(part 1 of 2)
# Autodesk Inventor assembly: Raspberry Pi 3
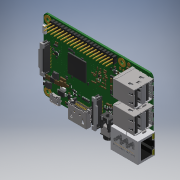
[picture p0: Inventor's stored thumbnail of the model, 180x180]
Saved by Autodesk Inventor 2017 (Build 210142000, 142)
## iProperties
Created: 2016-07-31
Part Number: Raspberry Pi 3
Document SubType Name: Assembly
Designer: jferner
Author: jferner
Sending System: SolidWorks 2016
Last Author: awillame
Last Saved: 2017-12-17
## Documents named in this file (329)
- C:\Users\jferner\Downloads\raspberry-pi-3-model-b-reference-design-solidworks-cad-rpi-raspberrypi-raspberry-pi-1.snapshot.83\Solidworks Complete Assembly\Raspberry Pi 3.iam
- C:\Users\jferner\Downloads\raspberry-pi-3-model-b-reference-design-solidworks-cad-rpi-raspberrypi-raspberry-pi-1.snapshot.83\Solidworks Complete Assembly\Raspberry Pi 3157.ipt
- C:\Users\jferner\Downloads\raspberry-pi-3-model-b-reference-design-solidworks-cad-rpi-raspberrypi-raspberry-pi-1.snapshot.83\Solidworks Complete Assembly\Raspberry Pi 3242.ipt
- C:\Users\jferner\Downloads\raspberry-pi-3-model-b-reference-design-solidworks-cad-rpi-raspberrypi-raspberry-pi-1.snapshot.83\Solidworks Complete Assembly\Raspberry Pi 3266.ipt
- C:\Users\jferner\Downloads\raspberry-pi-3-model-b-reference-design-solidworks-cad-rpi-raspberrypi-raspberry-pi-1.snapshot.83\Solidworks Complete Assembly\raspberry_pi_3(bar_180_2x20).ipt
- C:\Users\jferner\Downloads\raspberry-pi-3-model-b-reference-design-solidworks-cad-rpi-raspberrypi-raspberry-pi-1.snapshot.83\Solidworks Complete Assembly\RPi3_ModelB v1.iam
- C:\Users\jferner\Downloads\raspberry-pi-3-model-b-reference-design-solidworks-cad-rpi-raspberrypi-raspberry-pi-1.snapshot.83\Solidworks Complete Assembly\Raspberry Pi 312.ipt
- C:\Users\jferner\Downloads\raspberry-pi-3-model-b-reference-design-solidworks-cad-rpi-raspberrypi-raspberry-pi-1.snapshot.83\Solidworks Complete Assembly\Raspberry Pi 314.ipt
- C:\Users\jferner\Downloads\raspberry-pi-3-model-b-reference-design-solidworks-cad-rpi-raspberrypi-raspberry-pi-1.snapshot.83\Solidworks Complete Assembly\Raspberry Pi 3172.ipt
- C:\Users\jferner\Downloads\raspberry-pi-3-model-b-reference-design-solidworks-cad-rpi-raspberrypi-raspberry-pi-1.snapshot.83\Solidworks Complete Assembly\Raspberry Pi 3173.ipt
- C:\Users\jferner\Downloads\raspberry-pi-3-model-b-reference-design-solidworks-cad-rpi-raspberrypi-raspberry-pi-1.snapshot.83\Solidworks Complete Assembly\Raspberry Pi 3174.ipt
- C:\Users\jferner\Downloads\raspberry-pi-3-model-b-reference-design-solidworks-cad-rpi-raspberrypi-raspberry-pi-1.snapshot.83\Solidworks Complete Assembly\Raspberry Pi 3175.ipt
- C:\Users\jferner\Downloads\raspberry-pi-3-model-b-reference-design-solidworks-cad-rpi-raspberrypi-raspberry-pi-1.snapshot.83\Solidworks Complete Assembly\Raspberry Pi 3176.ipt
- C:\Users\jferner\Downloads\raspberry-pi-3-model-b-reference-design-solidworks-cad-rpi-raspberrypi-raspberry-pi-1.snapshot.83\Solidworks Complete Assembly\Raspberry Pi 3177.ipt
- C:\Users\jferner\Downloads\raspberry-pi-3-model-b-reference-design-solidworks-cad-rpi-raspberrypi-raspberry-pi-1.snapshot.83\Solidworks Complete Assembly\Raspberry Pi 3178.ipt
- C:\Users\jferner\Downloads\raspberry-pi-3-model-b-reference-design-solidworks-cad-rpi-raspberrypi-raspberry-pi-1.snapshot.83\Solidworks Complete Assembly\Raspberry Pi 3179.ipt
- C:\Users\jferner\Downloads\raspberry-pi-3-model-b-reference-design-solidworks-cad-rpi-raspberrypi-raspberry-pi-1.snapshot.83\Solidworks Complete Assembly\Raspberry Pi 3180.ipt
- C:\Users\jferner\Downloads\raspberry-pi-3-model-b-reference-design-solidworks-cad-rpi-raspberrypi-raspberry-pi-1.snapshot.83\Solidworks Complete Assembly\Raspberry Pi 3181.ipt
- C:\Users\jferner\Downloads\raspberry-pi-3-model-b-reference-design-solidworks-cad-rpi-raspberrypi-raspberry-pi-1.snapshot.83\Solidworks Complete Assembly\Raspberry Pi 3182.ipt
- C:\Users\jferner\Downloads\raspberry-pi-3-model-b-reference-design-solidworks-cad-rpi-raspberrypi-raspberry-pi-1.snapshot.83\Solidworks Complete Assembly\Raspberry Pi 3183.ipt
- C:\Users\jferner\Downloads\raspberry-pi-3-model-b-reference-design-solidworks-cad-rpi-raspberrypi-raspberry-pi-1.snapshot.83\Solidworks Complete Assembly\Raspberry Pi 3184.ipt
- C:\Users\jferner\Downloads\raspberry-pi-3-model-b-reference-design-solidworks-cad-rpi-raspberrypi-raspberry-pi-1.snapshot.83\Solidworks Complete Assembly\Raspberry Pi 3185.ipt
- C:\Users\jferner\Downloads\raspberry-pi-3-model-b-reference-design-solidworks-cad-rpi-raspberrypi-raspberry-pi-1.snapshot.83\Solidworks Complete Assembly\Raspberry Pi 3186.ipt
- C:\Users\jferner\Downloads\raspberry-pi-3-model-b-reference-design-solidworks-cad-rpi-raspberrypi-raspberry-pi-1.snapshot.83\Solidworks Complete Assembly\Raspberry Pi 3187.ipt
- C:\Users\jferner\Downloads\raspberry-pi-3-model-b-reference-design-solidworks-cad-rpi-raspberrypi-raspberry-pi-1.snapshot.83\Solidworks Complete Assembly\Raspberry Pi 3188.ipt
- C:\Users\jferner\Downloads\raspberry-pi-3-model-b-reference-design-solidworks-cad-rpi-raspberrypi-raspberry-pi-1.snapshot.83\Solidworks Complete Assembly\Raspberry Pi 3189.ipt
- C:\Users\jferner\Downloads\raspberry-pi-3-model-b-reference-design-solidworks-cad-rpi-raspberrypi-raspberry-pi-1.snapshot.83\Solidworks Complete Assembly\Raspberry Pi 3190.ipt
- C:\Users\jferner\Downloads\raspberry-pi-3-model-b-reference-design-solidworks-cad-rpi-raspberrypi-raspberry-pi-1.snapshot.83\Solidworks Complete Assembly\Raspberry Pi 3191.ipt
- C:\Users\jferner\Downloads\raspberry-pi-3-model-b-reference-design-solidworks-cad-rpi-raspberrypi-raspberry-pi-1.snapshot.83\Solidworks Complete Assembly\Raspberry Pi 3192.ipt
- C:\Users\jferner\Downloads\raspberry-pi-3-model-b-reference-design-solidworks-cad-rpi-raspberrypi-raspberry-pi-1.snapshot.83\Solidworks Complete Assembly\Raspberry Pi 3193.ipt
- C:\Users\jferner\Downloads\raspberry-pi-3-model-b-reference-design-solidworks-cad-rpi-raspberrypi-raspberry-pi-1.snapshot.83\Solidworks Complete Assembly\Raspberry Pi 3194.ipt
- C:\Users\jferner\Downloads\raspberry-pi-3-model-b-reference-design-solidworks-cad-rpi-raspberrypi-raspberry-pi-1.snapshot.83\Solidworks Complete Assembly\Raspberry Pi 3195.ipt
- C:\Users\jferner\Downloads\raspberry-pi-3-model-b-reference-design-solidworks-cad-rpi-raspberrypi-raspberry-pi-1.snapshot.83\Solidworks Complete Assembly\Raspberry Pi 3196.ipt
- C:\Users\jferner\Downloads\raspberry-pi-3-model-b-reference-design-solidworks-cad-rpi-raspberrypi-raspberry-pi-1.snapshot.83\Solidworks Complete Assembly\Raspberry Pi 3197.ipt
- C:\Users\jferner\Downloads\raspberry-pi-3-model-b-reference-design-solidworks-cad-rpi-raspberrypi-raspberry-pi-1.snapshot.83\Solidworks Complete Assembly\Raspberry Pi 3198.ipt
- C:\Users\jferner\Downloads\raspberry-pi-3-model-b-reference-design-solidworks-cad-rpi-raspberrypi-raspberry-pi-1.snapshot.83\Solidworks Complete Assembly\Raspberry Pi 3199.ipt
- C:\Users\jferner\Downloads\raspberry-pi-3-model-b-reference-design-solidworks-cad-rpi-raspberrypi-raspberry-pi-1.snapshot.83\Solidworks Complete Assembly\Raspberry Pi 3200.ipt
- C:\Users\jferner\Downloads\raspberry-pi-3-model-b-reference-design-solidworks-cad-rpi-raspberrypi-raspberry-pi-1.snapshot.83\Solidworks Complete Assembly\Raspberry Pi 3201.ipt
- C:\Users\jferner\Downloads\raspberry-pi-3-model-b-reference-design-solidworks-cad-rpi-raspberrypi-raspberry-pi-1.snapshot.83\Solidworks Complete Assembly\Raspberry Pi 3202.ipt
- C:\Users\jferner\Downloads\raspberry-pi-3-model-b-reference-design-solidworks-cad-rpi-raspberrypi-raspberry-pi-1.snapshot.83\Solidworks Complete Assembly\Raspberry Pi 3203.ipt
- C:\Users\jferner\Downloads\raspberry-pi-3-model-b-reference-design-solidworks-cad-rpi-raspberrypi-raspberry-pi-1.snapshot.83\Solidworks Complete Assembly\Raspberry Pi 3204.ipt
- C:\Users\jferner\Downloads\raspberry-pi-3-model-b-reference-design-solidworks-cad-rpi-raspberrypi-raspberry-pi-1.snapshot.83\Solidworks Complete Assembly\Raspberry Pi 3205.ipt
- C:\Users\jferner\Downloads\raspberry-pi-3-model-b-reference-design-solidworks-cad-rpi-raspberrypi-raspberry-pi-1.snapshot.83\Solidworks Complete Assembly\Raspberry Pi 3206.ipt
- C:\Users\jferner\Downloads\raspberry-pi-3-model-b-reference-design-solidworks-cad-rpi-raspberrypi-raspberry-pi-1.snapshot.83\Solidworks Complete Assembly\Raspberry Pi 3207.ipt
- C:\Users\jferner\Downloads\raspberry-pi-3-model-b-reference-design-solidworks-cad-rpi-raspberrypi-raspberry-pi-1.snapshot.83\Solidworks Complete Assembly\Raspberry Pi 3208.ipt
- C:\Users\jferner\Downloads\raspberry-pi-3-model-b-reference-design-solidworks-cad-rpi-raspberrypi-raspberry-pi-1.snapshot.83\Solidworks Complete Assembly\Raspberry Pi 3209.ipt
- C:\Users\jferner\Downloads\raspberry-pi-3-model-b-reference-design-solidworks-cad-rpi-raspberrypi-raspberry-pi-1.snapshot.83\Solidworks Complete Assembly\Raspberry Pi 3210.ipt
- C:\Users\jferner\Downloads\raspberry-pi-3-model-b-reference-design-solidworks-cad-rpi-raspberrypi-raspberry-pi-1.snapshot.83\Solidworks Complete Assembly\Raspberry Pi 3211.ipt
- C:\Users\jferner\Downloads\raspberry-pi-3-model-b-reference-design-solidworks-cad-rpi-raspberrypi-raspberry-pi-1.snapshot.83\Solidworks Complete Assembly\Raspberry Pi 3212.ipt
- C:\Users\jferner\Downloads\raspberry-pi-3-model-b-reference-design-solidworks-cad-rpi-raspberrypi-raspberry-pi-1.snapshot.83\Solidworks Complete Assembly\Raspberry Pi 3213.ipt
- C:\Users\jferner\Downloads\raspberry-pi-3-model-b-reference-design-solidworks-cad-rpi-raspberrypi-raspberry-pi-1.snapshot.83\Solidworks Complete Assembly\Raspberry Pi 3214.ipt
- C:\Users\jferner\Downloads\raspberry-pi-3-model-b-reference-design-solidworks-cad-rpi-raspberrypi-raspberry-pi-1.snapshot.83\Solidworks Complete Assembly\Raspberry Pi 3215.ipt
- C:\Users\jferner\Downloads\raspberry-pi-3-model-b-reference-design-solidworks-cad-rpi-raspberrypi-raspberry-pi-1.snapshot.83\Solidworks Complete Assembly\Raspberry Pi 3216.ipt
- C:\Users\jferner\Downloads\raspberry-pi-3-model-b-reference-design-solidworks-cad-rpi-raspberrypi-raspberry-pi-1.snapshot.83\Solidworks Complete Assembly\Raspberry Pi 3217.ipt
- C:\Users\jferner\Downloads\raspberry-pi-3-model-b-reference-design-solidworks-cad-rpi-raspberrypi-raspberry-pi-1.snapshot.83\Solidworks Complete Assembly\Raspberry Pi 3218.ipt
- C:\Users\jferner\Downloads\raspberry-pi-3-model-b-reference-design-solidworks-cad-rpi-raspberrypi-raspberry-pi-1.snapshot.83\Solidworks Complete Assembly\Raspberry Pi 3219.ipt
- C:\Users\jferner\Downloads\raspberry-pi-3-model-b-reference-design-solidworks-cad-rpi-raspberrypi-raspberry-pi-1.snapshot.83\Solidworks Complete Assembly\Raspberry Pi 3220.ipt
- C:\Users\jferner\Downloads\raspberry-pi-3-model-b-reference-design-solidworks-cad-rpi-raspberrypi-raspberry-pi-1.snapshot.83\Solidworks Complete Assembly\Raspberry Pi 3221.ipt
- C:\Users\jferner\Downloads\raspberry-pi-3-model-b-reference-design-solidworks-cad-rpi-raspberrypi-raspberry-pi-1.snapshot.83\Solidworks Complete Assembly\Raspberry Pi 3222.ipt
- C:\Users\jferner\Downloads\raspberry-pi-3-model-b-reference-design-solidworks-cad-rpi-raspberrypi-raspberry-pi-1.snapshot.83\Solidworks Complete Assembly\Raspberry Pi 3223.ipt
- C:\Users\jferner\Downloads\raspberry-pi-3-model-b-reference-design-solidworks-cad-rpi-raspberrypi-raspberry-pi-1.snapshot.83\Solidworks Complete Assembly\Raspberry Pi 3224.ipt
- C:\Users\jferner\Downloads\raspberry-pi-3-model-b-reference-design-solidworks-cad-rpi-raspberrypi-raspberry-pi-1.snapshot.83\Solidworks Complete Assembly\Raspberry Pi 3225.ipt
- C:\Users\jferner\Downloads\raspberry-pi-3-model-b-reference-design-solidworks-cad-rpi-raspberrypi-raspberry-pi-1.snapshot.83\Solidworks Complete Assembly\Raspberry Pi 3226.ipt
- C:\Users\jferner\Downloads\raspberry-pi-3-model-b-reference-design-solidworks-cad-rpi-raspberrypi-raspberry-pi-1.snapshot.83\Solidworks Complete Assembly\Raspberry Pi 3227.ipt
- C:\Users\jferner\Downloads\raspberry-pi-3-model-b-reference-design-solidworks-cad-rpi-raspberrypi-raspberry-pi-1.snapshot.83\Solidworks Complete Assembly\Raspberry Pi 3228.ipt
- C:\Users\jferner\Downloads\raspberry-pi-3-model-b-reference-design-solidworks-cad-rpi-raspberrypi-raspberry-pi-1.snapshot.83\Solidworks Complete Assembly\Raspberry Pi 3229.ipt
- C:\Users\jferner\Downloads\raspberry-pi-3-model-b-reference-design-solidworks-cad-rpi-raspberrypi-raspberry-pi-1.snapshot.83\Solidworks Complete Assembly\Raspberry Pi 3230.ipt
- C:\Users\jferner\Downloads\raspberry-pi-3-model-b-reference-design-solidworks-cad-rpi-raspberrypi-raspberry-pi-1.snapshot.83\Solidworks Complete Assembly\Raspberry Pi 3231.ipt
- C:\Users\jferner\Downloads\raspberry-pi-3-model-b-reference-design-solidworks-cad-rpi-raspberrypi-raspberry-pi-1.snapshot.83\Solidworks Complete Assembly\Raspberry Pi 3232.ipt
- C:\Users\jferner\Downloads\raspberry-pi-3-model-b-reference-design-solidworks-cad-rpi-raspberrypi-raspberry-pi-1.snapshot.83\Solidworks Complete Assembly\Raspberry Pi 3233.ipt
- C:\Users\jferner\Downloads\raspberry-pi-3-model-b-reference-design-solidworks-cad-rpi-raspberrypi-raspberry-pi-1.snapshot.83\Solidworks Complete Assembly\Raspberry Pi 3234.ipt
- C:\Users\jferner\Downloads\raspberry-pi-3-model-b-reference-design-solidworks-cad-rpi-raspberrypi-raspberry-pi-1.snapshot.83\Solidworks Complete Assembly\Raspberry Pi 3235.ipt
- C:\Users\jferner\Downloads\raspberry-pi-3-model-b-reference-design-solidworks-cad-rpi-raspberrypi-raspberry-pi-1.snapshot.83\Solidworks Complete Assembly\Raspberry Pi 31.ipt
- C:\Users\jferner\Downloads\raspberry-pi-3-model-b-reference-design-solidworks-cad-rpi-raspberrypi-raspberry-pi-1.snapshot.83\Solidworks Complete Assembly\Raspberry Pi 36.ipt
- C:\Users\jferner\Downloads\raspberry-pi-3-model-b-reference-design-solidworks-cad-rpi-raspberrypi-raspberry-pi-1.snapshot.83\Solidworks Complete Assembly\Raspberry Pi 32.ipt
- C:\Users\jferner\Downloads\raspberry-pi-3-model-b-reference-design-solidworks-cad-rpi-raspberrypi-raspberry-pi-1.snapshot.83\Solidworks Complete Assembly\Raspberry Pi 33.ipt
- C:\Users\jferner\Downloads\raspberry-pi-3-model-b-reference-design-solidworks-cad-rpi-raspberrypi-raspberry-pi-1.snapshot.83\Solidworks Complete Assembly\Raspberry Pi 34.ipt
- C:\Users\jferner\Downloads\raspberry-pi-3-model-b-reference-design-solidworks-cad-rpi-raspberrypi-raspberry-pi-1.snapshot.83\Solidworks Complete Assembly\Raspberry Pi 35.ipt
- C:\Users\jferner\Downloads\raspberry-pi-3-model-b-reference-design-solidworks-cad-rpi-raspberrypi-raspberry-pi-1.snapshot.83\Solidworks Complete Assembly\Raspberry Pi 37.ipt
- C:\Users\jferner\Downloads\raspberry-pi-3-model-b-reference-design-solidworks-cad-rpi-raspberrypi-raspberry-pi-1.snapshot.83\Solidworks Complete Assembly\Raspberry Pi 38.ipt
- C:\Users\jferner\Downloads\raspberry-pi-3-model-b-reference-design-solidworks-cad-rpi-raspberrypi-raspberry-pi-1.snapshot.83\Solidworks Complete Assembly\Raspberry Pi 39.ipt
- C:\Users\jferner\Downloads\raspberry-pi-3-model-b-reference-design-solidworks-cad-rpi-raspberrypi-raspberry-pi-1.snapshot.83\Solidworks Complete Assembly\Raspberry Pi 310.ipt
- C:\Users\jferner\Downloads\raspberry-pi-3-model-b-reference-design-solidworks-cad-rpi-raspberrypi-raspberry-pi-1.snapshot.83\Solidworks Complete Assembly\Raspberry Pi 311.ipt
- C:\Users\jferner\Downloads\raspberry-pi-3-model-b-reference-design-solidworks-cad-rpi-raspberrypi-raspberry-pi-1.snapshot.83\Solidworks Complete Assembly\Raspberry Pi 313.ipt
- C:\Users\jferner\Downloads\raspberry-pi-3-model-b-reference-design-solidworks-cad-rpi-raspberrypi-raspberry-pi-1.snapshot.83\Solidworks Complete Assembly\Raspberry Pi 315.ipt
- C:\Users\jferner\Downloads\raspberry-pi-3-model-b-reference-design-solidworks-cad-rpi-raspberrypi-raspberry-pi-1.snapshot.83\Solidworks Complete Assembly\Raspberry Pi 316.ipt
- C:\Users\jferner\Downloads\raspberry-pi-3-model-b-reference-design-solidworks-cad-rpi-raspberrypi-raspberry-pi-1.snapshot.83\Solidworks Complete Assembly\Raspberry Pi 317.ipt
- C:\Users\jferner\Downloads\raspberry-pi-3-model-b-reference-design-solidworks-cad-rpi-raspberrypi-raspberry-pi-1.snapshot.83\Solidworks Complete Assembly\Raspberry Pi 318.ipt
- C:\Users\jferner\Downloads\raspberry-pi-3-model-b-reference-design-solidworks-cad-rpi-raspberrypi-raspberry-pi-1.snapshot.83\Solidworks Complete Assembly\Raspberry Pi 319.ipt
- C:\Users\jferner\Downloads\raspberry-pi-3-model-b-reference-design-solidworks-cad-rpi-raspberrypi-raspberry-pi-1.snapshot.83\Solidworks Complete Assembly\Raspberry Pi 320.ipt
- C:\Users\jferner\Downloads\raspberry-pi-3-model-b-reference-design-solidworks-cad-rpi-raspberrypi-raspberry-pi-1.snapshot.83\Solidworks Complete Assembly\Raspberry Pi 322.ipt
- C:\Users\jferner\Downloads\raspberry-pi-3-model-b-reference-design-solidworks-cad-rpi-raspberrypi-raspberry-pi-1.snapshot.83\Solidworks Complete Assembly\Raspberry Pi 323.ipt
- C:\Users\jferner\Downloads\raspberry-pi-3-model-b-reference-design-solidworks-cad-rpi-raspberrypi-raspberry-pi-1.snapshot.83\Solidworks Complete Assembly\Raspberry Pi 324.ipt
- C:\Users\jferner\Downloads\raspberry-pi-3-model-b-reference-design-solidworks-cad-rpi-raspberrypi-raspberry-pi-1.snapshot.83\Solidworks Complete Assembly\Raspberry Pi 325.ipt
- C:\Users\jferner\Downloads\raspberry-pi-3-model-b-reference-design-solidworks-cad-rpi-raspberrypi-raspberry-pi-1.snapshot.83\Solidworks Complete Assembly\Raspberry Pi 326.ipt
- C:\Users\jferner\Downloads\raspberry-pi-3-model-b-reference-design-solidworks-cad-rpi-raspberrypi-raspberry-pi-1.snapshot.83\Solidworks Complete Assembly\Raspberry Pi 327.ipt
- C:\Users\jferner\Downloads\raspberry-pi-3-model-b-reference-design-solidworks-cad-rpi-raspberrypi-raspberry-pi-1.snapshot.83\Solidworks Complete Assembly\Raspberry Pi 328.ipt
- C:\Users\jferner\Downloads\raspberry-pi-3-model-b-reference-design-solidworks-cad-rpi-raspberrypi-raspberry-pi-1.snapshot.83\Solidworks Complete Assembly\Raspberry Pi 329.ipt
- C:\Users\jferner\Downloads\raspberry-pi-3-model-b-reference-design-solidworks-cad-rpi-raspberrypi-raspberry-pi-1.snapshot.83\Solidworks Complete Assembly\Raspberry Pi 330.ipt
- C:\Users\jferner\Downloads\raspberry-pi-3-model-b-reference-design-solidworks-cad-rpi-raspberrypi-raspberry-pi-1.snapshot.83\Solidworks Complete Assembly\Raspberry Pi 331.ipt
- C:\Users\jferner\Downloads\raspberry-pi-3-model-b-reference-design-solidworks-cad-rpi-raspberrypi-raspberry-pi-1.snapshot.83\Solidworks Complete Assembly\Raspberry Pi 332.ipt
- C:\Users\jferner\Downloads\raspberry-pi-3-model-b-reference-design-solidworks-cad-rpi-raspberrypi-raspberry-pi-1.snapshot.83\Solidworks Complete Assembly\Raspberry Pi 333.ipt
- C:\Users\jferner\Downloads\raspberry-pi-3-model-b-reference-design-solidworks-cad-rpi-raspberrypi-raspberry-pi-1.snapshot.83\Solidworks Complete Assembly\Raspberry Pi 334.ipt
- C:\Users\jferner\Downloads\raspberry-pi-3-model-b-reference-design-solidworks-cad-rpi-raspberrypi-raspberry-pi-1.snapshot.83\Solidworks Complete Assembly\Raspberry Pi 335.ipt
- C:\Users\jferner\Downloads\raspberry-pi-3-model-b-reference-design-solidworks-cad-rpi-raspberrypi-raspberry-pi-1.snapshot.83\Solidworks Complete Assembly\Raspberry Pi 336.ipt
- C:\Users\jferner\Downloads\raspberry-pi-3-model-b-reference-design-solidworks-cad-rpi-raspberrypi-raspberry-pi-1.snapshot.83\Solidworks Complete Assembly\Raspberry Pi 337.ipt
- C:\Users\jferner\Downloads\raspberry-pi-3-model-b-reference-design-solidworks-cad-rpi-raspberrypi-raspberry-pi-1.snapshot.83\Solidworks Complete Assembly\Raspberry Pi 338.ipt
- C:\Users\jferner\Downloads\raspberry-pi-3-model-b-reference-design-solidworks-cad-rpi-raspberrypi-raspberry-pi-1.snapshot.83\Solidworks Complete Assembly\Raspberry Pi 339.ipt
- C:\Users\jferner\Downloads\raspberry-pi-3-model-b-reference-design-solidworks-cad-rpi-raspberrypi-raspberry-pi-1.snapshot.83\Solidworks Complete Assembly\Raspberry Pi 340.ipt
- C:\Users\jferner\Downloads\raspberry-pi-3-model-b-reference-design-solidworks-cad-rpi-raspberrypi-raspberry-pi-1.snapshot.83\Solidworks Complete Assembly\Raspberry Pi 341.ipt
- C:\Users\jferner\Downloads\raspberry-pi-3-model-b-reference-design-solidworks-cad-rpi-raspberrypi-raspberry-pi-1.snapshot.83\Solidworks Complete Assembly\Raspberry Pi 342.ipt
- C:\Users\jferner\Downloads\raspberry-pi-3-model-b-reference-design-solidworks-cad-rpi-raspberrypi-raspberry-pi-1.snapshot.83\Solidworks Complete Assembly\Raspberry Pi 343.ipt
- C:\Users\jferner\Downloads\raspberry-pi-3-model-b-reference-design-solidworks-cad-rpi-raspberrypi-raspberry-pi-1.snapshot.83\Solidworks Complete Assembly\Raspberry Pi 344.ipt
- C:\Users\jferner\Downloads\raspberry-pi-3-model-b-reference-design-solidworks-cad-rpi-raspberrypi-raspberry-pi-1.snapshot.83\Solidworks Complete Assembly\Raspberry Pi 345.ipt
- C:\Users\jferner\Downloads\raspberry-pi-3-model-b-reference-design-solidworks-cad-rpi-raspberrypi-raspberry-pi-1.snapshot.83\Solidworks Complete Assembly\Raspberry Pi 346.ipt
- C:\Users\jferner\Downloads\raspberry-pi-3-model-b-reference-design-solidworks-cad-rpi-raspberrypi-raspberry-pi-1.snapshot.83\Solidworks Complete Assembly\Raspberry Pi 347.ipt
- C:\Users\jferner\Downloads\raspberry-pi-3-model-b-reference-design-solidworks-cad-rpi-raspberrypi-raspberry-pi-1.snapshot.83\Solidworks Complete Assembly\Raspberry Pi 348.ipt
- C:\Users\jferner\Downloads\raspberry-pi-3-model-b-reference-design-solidworks-cad-rpi-raspberrypi-raspberry-pi-1.snapshot.83\Solidworks Complete Assembly\Raspberry Pi 349.ipt
- C:\Users\jferner\Downloads\raspberry-pi-3-model-b-reference-design-solidworks-cad-rpi-raspberrypi-raspberry-pi-1.snapshot.83\Solidworks Complete Assembly\Raspberry Pi 350.ipt
- C:\Users\jferner\Downloads\raspberry-pi-3-model-b-reference-design-solidworks-cad-rpi-raspberrypi-raspberry-pi-1.snapshot.83\Solidworks Complete Assembly\Raspberry Pi 351.ipt
- C:\Users\jferner\Downloads\raspberry-pi-3-model-b-reference-design-solidworks-cad-rpi-raspberrypi-raspberry-pi-1.snapshot.83\Solidworks Complete Assembly\Raspberry Pi 352.ipt
- C:\Users\jferner\Downloads\raspberry-pi-3-model-b-reference-design-solidworks-cad-rpi-raspberrypi-raspberry-pi-1.snapshot.83\Solidworks Complete Assembly\Raspberry Pi 353.ipt
- C:\Users\jferner\Downloads\raspberry-pi-3-model-b-reference-design-solidworks-cad-rpi-raspberrypi-raspberry-pi-1.snapshot.83\Solidworks Complete Assembly\Raspberry Pi 354.ipt
- C:\Users\jferner\Downloads\raspberry-pi-3-model-b-reference-design-solidworks-cad-rpi-raspberrypi-raspberry-pi-1.snapshot.83\Solidworks Complete Assembly\Raspberry Pi 355.ipt
- C:\Users\jferner\Downloads\raspberry-pi-3-model-b-reference-design-solidworks-cad-rpi-raspberrypi-raspberry-pi-1.snapshot.83\Solidworks Complete Assembly\Raspberry Pi 356.ipt
- C:\Users\jferner\Downloads\raspberry-pi-3-model-b-reference-design-solidworks-cad-rpi-raspberrypi-raspberry-pi-1.snapshot.83\Solidworks Complete Assembly\Raspberry Pi 357.ipt
- C:\Users\jferner\Downloads\raspberry-pi-3-model-b-reference-design-solidworks-cad-rpi-raspberrypi-raspberry-pi-1.snapshot.83\Solidworks Complete Assembly\Raspberry Pi 358.ipt
- C:\Users\jferner\Downloads\raspberry-pi-3-model-b-reference-design-solidworks-cad-rpi-raspberrypi-raspberry-pi-1.snapshot.83\Solidworks Complete Assembly\Raspberry Pi 359.ipt
- C:\Users\jferner\Downloads\raspberry-pi-3-model-b-reference-design-solidworks-cad-rpi-raspberrypi-raspberry-pi-1.snapshot.83\Solidworks Complete Assembly\Raspberry Pi 360.ipt
- C:\Users\jferner\Downloads\raspberry-pi-3-model-b-reference-design-solidworks-cad-rpi-raspberrypi-raspberry-pi-1.snapshot.83\Solidworks Complete Assembly\Raspberry Pi 361.ipt
- C:\Users\jferner\Downloads\raspberry-pi-3-model-b-reference-design-solidworks-cad-rpi-raspberrypi-raspberry-pi-1.snapshot.83\Solidworks Complete Assembly\Raspberry Pi 362.ipt
- C:\Users\jferner\Downloads\raspberry-pi-3-model-b-reference-design-solidworks-cad-rpi-raspberrypi-raspberry-pi-1.snapshot.83\Solidworks Complete Assembly\Raspberry Pi 363.ipt
- C:\Users\jferner\Downloads\raspberry-pi-3-model-b-reference-design-solidworks-cad-rpi-raspberrypi-raspberry-pi-1.snapshot.83\Solidworks Complete Assembly\Raspberry Pi 364.ipt
- C:\Users\jferner\Downloads\raspberry-pi-3-model-b-reference-design-solidworks-cad-rpi-raspberrypi-raspberry-pi-1.snapshot.83\Solidworks Complete Assembly\Raspberry Pi 365.ipt
- C:\Users\jferner\Downloads\raspberry-pi-3-model-b-reference-design-solidworks-cad-rpi-raspberrypi-raspberry-pi-1.snapshot.83\Solidworks Complete Assembly\Raspberry Pi 366.ipt
- C:\Users\jferner\Downloads\raspberry-pi-3-model-b-reference-design-solidworks-cad-rpi-raspberrypi-raspberry-pi-1.snapshot.83\Solidworks Complete Assembly\Raspberry Pi 367.ipt
- C:\Users\jferner\Downloads\raspberry-pi-3-model-b-reference-design-solidworks-cad-rpi-raspberrypi-raspberry-pi-1.snapshot.83\Solidworks Complete Assembly\Raspberry Pi 368.ipt
- C:\Users\jferner\Downloads\raspberry-pi-3-model-b-reference-design-solidworks-cad-rpi-raspberrypi-raspberry-pi-1.snapshot.83\Solidworks Complete Assembly\Raspberry Pi 369.ipt
- C:\Users\jferner\Downloads\raspberry-pi-3-model-b-reference-design-solidworks-cad-rpi-raspberrypi-raspberry-pi-1.snapshot.83\Solidworks Complete Assembly\Raspberry Pi 370.ipt
- C:\Users\jferner\Downloads\raspberry-pi-3-model-b-reference-design-solidworks-cad-rpi-raspberrypi-raspberry-pi-1.snapshot.83\Solidworks Complete Assembly\Raspberry Pi 371.ipt
- C:\Users\jferner\Downloads\raspberry-pi-3-model-b-reference-design-solidworks-cad-rpi-raspberrypi-raspberry-pi-1.snapshot.83\Solidworks Complete Assembly\Raspberry Pi 372.ipt
- C:\Users\jferner\Downloads\raspberry-pi-3-model-b-reference-design-solidworks-cad-rpi-raspberrypi-raspberry-pi-1.snapshot.83\Solidworks Complete Assembly\Raspberry Pi 373.ipt
- C:\Users\jferner\Downloads\raspberry-pi-3-model-b-reference-design-solidworks-cad-rpi-raspberrypi-raspberry-pi-1.snapshot.83\Solidworks Complete Assembly\Raspberry Pi 374.ipt
- C:\Users\jferner\Downloads\raspberry-pi-3-model-b-reference-design-solidworks-cad-rpi-raspberrypi-raspberry-pi-1.snapshot.83\Solidworks Complete Assembly\Raspberry Pi 375.ipt
- C:\Users\jferner\Downloads\raspberry-pi-3-model-b-reference-design-solidworks-cad-rpi-raspberrypi-raspberry-pi-1.snapshot.83\Solidworks Complete Assembly\Raspberry Pi 376.ipt
- C:\Users\jferner\Downloads\raspberry-pi-3-model-b-reference-design-solidworks-cad-rpi-raspberrypi-raspberry-pi-1.snapshot.83\Solidworks Complete Assembly\Raspberry Pi 377.ipt
- C:\Users\jferner\Downloads\raspberry-pi-3-model-b-reference-design-solidworks-cad-rpi-raspberrypi-raspberry-pi-1.snapshot.83\Solidworks Complete Assembly\Raspberry Pi 378.ipt
- C:\Users\jferner\Downloads\raspberry-pi-3-model-b-reference-design-solidworks-cad-rpi-raspberrypi-raspberry-pi-1.snapshot.83\Solidworks Complete Assembly\Raspberry Pi 379.ipt
- C:\Users\jferner\Downloads\raspberry-pi-3-model-b-reference-design-solidworks-cad-rpi-raspberrypi-raspberry-pi-1.snapshot.83\Solidworks Complete Assembly\Raspberry Pi 380.ipt
- C:\Users\jferner\Downloads\raspberry-pi-3-model-b-reference-design-solidworks-cad-rpi-raspberrypi-raspberry-pi-1.snapshot.83\Solidworks Complete Assembly\Raspberry Pi 381.ipt
- C:\Users\jferner\Downloads\raspberry-pi-3-model-b-reference-design-solidworks-cad-rpi-raspberrypi-raspberry-pi-1.snapshot.83\Solidworks Complete Assembly\Raspberry Pi 382.ipt
- C:\Users\jferner\Downloads\raspberry-pi-3-model-b-reference-design-solidworks-cad-rpi-raspberrypi-raspberry-pi-1.snapshot.83\Solidworks Complete Assembly\Raspberry Pi 383.ipt
- C:\Users\jferner\Downloads\raspberry-pi-3-model-b-reference-design-solidworks-cad-rpi-raspberrypi-raspberry-pi-1.snapshot.83\Solidworks Complete Assembly\Raspberry Pi 385.ipt
- C:\Users\jferner\Downloads\raspberry-pi-3-model-b-reference-design-solidworks-cad-rpi-raspberrypi-raspberry-pi-1.snapshot.83\Solidworks Complete Assembly\Raspberry Pi 386.ipt
- C:\Users\jferner\Downloads\raspberry-pi-3-model-b-reference-design-solidworks-cad-rpi-raspberrypi-raspberry-pi-1.snapshot.83\Solidworks Complete Assembly\Raspberry Pi 387.ipt
- C:\Users\jferner\Downloads\raspberry-pi-3-model-b-reference-design-solidworks-cad-rpi-raspberrypi-raspberry-pi-1.snapshot.83\Solidworks Complete Assembly\Raspberry Pi 388.ipt
- C:\Users\jferner\Downloads\raspberry-pi-3-model-b-reference-design-solidworks-cad-rpi-raspberrypi-raspberry-pi-1.snapshot.83\Solidworks Complete Assembly\Raspberry Pi 390.ipt
- C:\Users\jferner\Downloads\raspberry-pi-3-model-b-reference-design-solidworks-cad-rpi-raspberrypi-raspberry-pi-1.snapshot.83\Solidworks Complete Assembly\Raspberry Pi 391.ipt
- C:\Users\jferner\Downloads\raspberry-pi-3-model-b-reference-design-solidworks-cad-rpi-raspberrypi-raspberry-pi-1.snapshot.83\Solidworks Complete Assembly\Raspberry Pi 393.ipt
- C:\Users\jferner\Downloads\raspberry-pi-3-model-b-reference-design-solidworks-cad-rpi-raspberrypi-raspberry-pi-1.snapshot.83\Solidworks Complete Assembly\Raspberry Pi 394.ipt
- C:\Users\jferner\Downloads\raspberry-pi-3-model-b-reference-design-solidworks-cad-rpi-raspberrypi-raspberry-pi-1.snapshot.83\Solidworks Complete Assembly\Raspberry Pi 395.ipt
- C:\Users\jferner\Downloads\raspberry-pi-3-model-b-reference-design-solidworks-cad-rpi-raspberrypi-raspberry-pi-1.snapshot.83\Solidworks Complete Assembly\Raspberry Pi 396.ipt
- C:\Users\jferner\Downloads\raspberry-pi-3-model-b-reference-design-solidworks-cad-rpi-raspberrypi-raspberry-pi-1.snapshot.83\Solidworks Complete Assembly\Raspberry Pi 397.ipt
- C:\Users\jferner\Downloads\raspberry-pi-3-model-b-reference-design-solidworks-cad-rpi-raspberrypi-raspberry-pi-1.snapshot.83\Solidworks Complete Assembly\Raspberry Pi 398.ipt
- C:\Users\jferner\Downloads\raspberry-pi-3-model-b-reference-design-solidworks-cad-rpi-raspberrypi-raspberry-pi-1.snapshot.83\Solidworks Complete Assembly\Raspberry Pi 399.ipt
- C:\Users\jferner\Downloads\raspberry-pi-3-model-b-reference-design-solidworks-cad-rpi-raspberrypi-raspberry-pi-1.snapshot.83\Solidworks Complete Assembly\Raspberry Pi 3100.ipt
- C:\Users\jferner\Downloads\raspberry-pi-3-model-b-reference-design-solidworks-cad-rpi-raspberrypi-raspberry-pi-1.snapshot.83\Solidworks Complete Assembly\Raspberry Pi 3101.ipt
- C:\Users\jferner\Downloads\raspberry-pi-3-model-b-reference-design-solidworks-cad-rpi-raspberrypi-raspberry-pi-1.snapshot.83\Solidworks Complete Assembly\Raspberry Pi 3102.ipt
- C:\Users\jferner\Downloads\raspberry-pi-3-model-b-reference-design-solidworks-cad-rpi-raspberrypi-raspberry-pi-1.snapshot.83\Solidworks Complete Assembly\Raspberry Pi 3103.ipt
- C:\Users\jferner\Downloads\raspberry-pi-3-model-b-reference-design-solidworks-cad-rpi-raspberrypi-raspberry-pi-1.snapshot.83\Solidworks Complete Assembly\Raspberry Pi 3104.ipt
- C:\Users\jferner\Downloads\raspberry-pi-3-model-b-reference-design-solidworks-cad-rpi-raspberrypi-raspberry-pi-1.snapshot.83\Solidworks Complete Assembly\Raspberry Pi 3105.ipt
- C:\Users\jferner\Downloads\raspberry-pi-3-model-b-reference-design-solidworks-cad-rpi-raspberrypi-raspberry-pi-1.snapshot.83\Solidworks Complete Assembly\Raspberry Pi 3106.ipt
- C:\Users\jferner\Downloads\raspberry-pi-3-model-b-reference-design-solidworks-cad-rpi-raspberrypi-raspberry-pi-1.snapshot.83\Solidworks Complete Assembly\Raspberry Pi 3107.ipt
- C:\Users\jferner\Downloads\raspberry-pi-3-model-b-reference-design-solidworks-cad-rpi-raspberrypi-raspberry-pi-1.snapshot.83\Solidworks Complete Assembly\Raspberry Pi 3108.ipt
- C:\Users\jferner\Downloads\raspberry-pi-3-model-b-reference-design-solidworks-cad-rpi-raspberrypi-raspberry-pi-1.snapshot.83\Solidworks Complete Assembly\Raspberry Pi 3109.ipt
- C:\Users\jferner\Downloads\raspberry-pi-3-model-b-reference-design-solidworks-cad-rpi-raspberrypi-raspberry-pi-1.snapshot.83\Solidworks Complete Assembly\Raspberry Pi 3110.ipt
- C:\Users\jferner\Downloads\raspberry-pi-3-model-b-reference-design-solidworks-cad-rpi-raspberrypi-raspberry-pi-1.snapshot.83\Solidworks Complete Assembly\Raspberry Pi 3111.ipt
- C:\Users\jferner\Downloads\raspberry-pi-3-model-b-reference-design-solidworks-cad-rpi-raspberrypi-raspberry-pi-1.snapshot.83\Solidworks Complete Assembly\Raspberry Pi 3112.ipt
- C:\Users\jferner\Downloads\raspberry-pi-3-model-b-reference-design-solidworks-cad-rpi-raspberrypi-raspberry-pi-1.snapshot.83\Solidworks Complete Assembly\Raspberry Pi 3113.ipt
- C:\Users\jferner\Downloads\raspberry-pi-3-model-b-reference-design-solidworks-cad-rpi-raspberrypi-raspberry-pi-1.snapshot.83\Solidworks Complete Assembly\Raspberry Pi 3114.ipt
- C:\Users\jferner\Downloads\raspberry-pi-3-model-b-reference-design-solidworks-cad-rpi-raspberrypi-raspberry-pi-1.snapshot.83\Solidworks Complete Assembly\Raspberry Pi 3115.ipt
- C:\Users\jferner\Downloads\raspberry-pi-3-model-b-reference-design-solidworks-cad-rpi-raspberrypi-raspberry-pi-1.snapshot.83\Solidworks Complete Assembly\Raspberry Pi 3116.ipt
- C:\Users\jferner\Downloads\raspberry-pi-3-model-b-reference-design-solidworks-cad-rpi-raspberrypi-raspberry-pi-1.snapshot.83\Solidworks Complete Assembly\Raspberry Pi 3117.ipt
- C:\Users\jferner\Downloads\raspberry-pi-3-model-b-reference-design-solidworks-cad-rpi-raspberrypi-raspberry-pi-1.snapshot.83\Solidworks Complete Assembly\Raspberry Pi 3118.ipt
- C:\Users\jferner\Downloads\raspberry-pi-3-model-b-reference-design-solidworks-cad-rpi-raspberrypi-raspberry-pi-1.snapshot.83\Solidworks Complete Assembly\Raspberry Pi 3119.ipt
- C:\Users\jferner\Downloads\raspberry-pi-3-model-b-reference-design-solidworks-cad-rpi-raspberrypi-raspberry-pi-1.snapshot.83\Solidworks Complete Assembly\Raspberry Pi 3120.ipt
- C:\Users\jferner\Downloads\raspberry-pi-3-model-b-reference-design-solidworks-cad-rpi-raspberrypi-raspberry-pi-1.snapshot.83\Solidworks Complete Assembly\Raspberry Pi 3121.ipt
- C:\Users\jferner\Downloads\raspberry-pi-3-model-b-reference-design-solidworks-cad-rpi-raspberrypi-raspberry-pi-1.snapshot.83\Solidworks Complete Assembly\Raspberry Pi 3122.ipt
- C:\Users\jferner\Downloads\raspberry-pi-3-model-b-reference-design-solidworks-cad-rpi-raspberrypi-raspberry-pi-1.snapshot.83\Solidworks Complete Assembly\Raspberry Pi 3123.ipt
- C:\Users\jferner\Downloads\raspberry-pi-3-model-b-reference-design-solidworks-cad-rpi-raspberrypi-raspberry-pi-1.snapshot.83\Solidworks Complete Assembly\Raspberry Pi 3124.ipt
- C:\Users\jferner\Downloads\raspberry-pi-3-model-b-reference-design-solidworks-cad-rpi-raspberrypi-raspberry-pi-1.snapshot.83\Solidworks Complete Assembly\Raspberry Pi 3125.ipt
- C:\Users\jferner\Downloads\raspberry-pi-3-model-b-reference-design-solidworks-cad-rpi-raspberrypi-raspberry-pi-1.snapshot.83\Solidworks Complete Assembly\Raspberry Pi 3126.ipt
- C:\Users\jferner\Downloads\raspberry-pi-3-model-b-reference-design-solidworks-cad-rpi-raspberrypi-raspberry-pi-1.snapshot.83\Solidworks Complete Assembly\Raspberry Pi 3127.ipt
- C:\Users\jferner\Downloads\raspberry-pi-3-model-b-reference-design-solidworks-cad-rpi-raspberrypi-raspberry-pi-1.snapshot.83\Solidworks Complete Assembly\Raspberry Pi 3128.ipt
- C:\Users\jferner\Downloads\raspberry-pi-3-model-b-reference-design-solidworks-cad-rpi-raspberrypi-raspberry-pi-1.snapshot.83\Solidworks Complete Assembly\Raspberry Pi 3129.ipt
- C:\Users\jferner\Downloads\raspberry-pi-3-model-b-reference-design-solidworks-cad-rpi-raspberrypi-raspberry-pi-1.snapshot.83\Solidworks Complete Assembly\Raspberry Pi 3130.ipt
- C:\Users\jferner\Downloads\raspberry-pi-3-model-b-reference-design-solidworks-cad-rpi-raspberrypi-raspberry-pi-1.snapshot.83\Solidworks Complete Assembly\Raspberry Pi 3131.ipt
- C:\Users\jferner\Downloads\raspberry-pi-3-model-b-reference-design-solidworks-cad-rpi-raspberrypi-raspberry-pi-1.snapshot.83\Solidworks Complete Assembly\Raspberry Pi 3132.ipt
- C:\Users\jferner\Downloads\raspberry-pi-3-model-b-reference-design-solidworks-cad-rpi-raspberrypi-raspberry-pi-1.snapshot.83\Solidworks Complete Assembly\Raspberry Pi 3133.ipt
- C:\Users\jferner\Downloads\raspberry-pi-3-model-b-reference-design-solidworks-cad-rpi-raspberrypi-raspberry-pi-1.snapshot.83\Solidworks Complete Assembly\Raspberry Pi 3134.ipt
- C:\Users\jferner\Downloads\raspberry-pi-3-model-b-reference-design-solidworks-cad-rpi-raspberrypi-raspberry-pi-1.snapshot.83\Solidworks Complete Assembly\Raspberry Pi 3135.ipt
- C:\Users\jferner\Downloads\raspberry-pi-3-model-b-reference-design-solidworks-cad-rpi-raspberrypi-raspberry-pi-1.snapshot.83\Solidworks Complete Assembly\Raspberry Pi 3137.ipt
- C:\Users\jferner\Downloads\raspberry-pi-3-model-b-reference-design-solidworks-cad-rpi-raspberrypi-raspberry-pi-1.snapshot.83\Solidworks Complete Assembly\Raspberry Pi 3138.ipt
- C:\Users\jferner\Downloads\raspberry-pi-3-model-b-reference-design-solidworks-cad-rpi-raspberrypi-raspberry-pi-1.snapshot.83\Solidworks Complete Assembly\Raspberry Pi 3139.ipt
- C:\Users\jferner\Downloads\raspberry-pi-3-model-b-reference-design-solidworks-cad-rpi-raspberrypi-raspberry-pi-1.snapshot.83\Solidworks Complete Assembly\Raspberry Pi 3140.ipt
- C:\Users\jferner\Downloads\raspberry-pi-3-model-b-reference-design-solidworks-cad-rpi-raspberrypi-raspberry-pi-1.snapshot.83\Solidworks Complete Assembly\Raspberry Pi 3141.ipt
- C:\Users\jferner\Downloads\raspberry-pi-3-model-b-reference-design-solidworks-cad-rpi-raspberrypi-raspberry-pi-1.snapshot.83\Solidworks Complete Assembly\Raspberry Pi 3142.ipt
- C:\Users\jferner\Downloads\raspberry-pi-3-model-b-reference-design-solidworks-cad-rpi-raspberrypi-raspberry-pi-1.snapshot.83\Solidworks Complete Assembly\Raspberry Pi 3143.ipt
- C:\Users\jferner\Downloads\raspberry-pi-3-model-b-reference-design-solidworks-cad-rpi-raspberrypi-raspberry-pi-1.snapshot.83\Solidworks Complete Assembly\Raspberry Pi 3144.ipt
- C:\Users\jferner\Downloads\raspberry-pi-3-model-b-reference-design-solidworks-cad-rpi-raspberrypi-raspberry-pi-1.snapshot.83\Solidworks Complete Assembly\Raspberry Pi 3146.ipt
- C:\Users\jferner\Downloads\raspberry-pi-3-model-b-reference-design-solidworks-cad-rpi-raspberrypi-raspberry-pi-1.snapshot.83\Solidworks Complete Assembly\Raspberry Pi 3147.ipt
- C:\Users\jferner\Downloads\raspberry-pi-3-model-b-reference-design-solidworks-cad-rpi-raspberrypi-raspberry-pi-1.snapshot.83\Solidworks Complete Assembly\Raspberry Pi 3149.ipt
- C:\Users\jferner\Downloads\raspberry-pi-3-model-b-reference-design-solidworks-cad-rpi-raspberrypi-raspberry-pi-1.snapshot.83\Solidworks Complete Assembly\Raspberry Pi 3150.ipt
- C:\Users\jferner\Downloads\raspberry-pi-3-model-b-reference-design-solidworks-cad-rpi-raspberrypi-raspberry-pi-1.snapshot.83\Solidworks Complete Assembly\Raspberry Pi 3151.ipt
- C:\Users\jferner\Downloads\raspberry-pi-3-model-b-reference-design-solidworks-cad-rpi-raspberrypi-raspberry-pi-1.snapshot.83\Solidworks Complete Assembly\Raspberry Pi 3152.ipt
- C:\Users\jferner\Downloads\raspberry-pi-3-model-b-reference-design-solidworks-cad-rpi-raspberrypi-raspberry-pi-1.snapshot.83\Solidworks Complete Assembly\Raspberry Pi 3153.ipt
- C:\Users\jferner\Downloads\raspberry-pi-3-model-b-reference-design-solidworks-cad-rpi-raspberrypi-raspberry-pi-1.snapshot.83\Solidworks Complete Assembly\Raspberry Pi 3154.ipt
- C:\Users\jferner\Downloads\raspberry-pi-3-model-b-reference-design-solidworks-cad-rpi-raspberrypi-raspberry-pi-1.snapshot.83\Solidworks Complete Assembly\Raspberry Pi 3155.ipt
- C:\Users\jferner\Downloads\raspberry-pi-3-model-b-reference-design-solidworks-cad-rpi-raspberrypi-raspberry-pi-1.snapshot.83\Solidworks Complete Assembly\Raspberry Pi 3156.ipt
- C:\Users\jferner\Downloads\raspberry-pi-3-model-b-reference-design-solidworks-cad-rpi-raspberrypi-raspberry-pi-1.snapshot.83\Solidworks Complete Assembly\Raspberry Pi 3158.ipt
- C:\Users\jferner\Downloads\raspberry-pi-3-model-b-reference-design-solidworks-cad-rpi-raspberrypi-raspberry-pi-1.snapshot.83\Solidworks Complete Assembly\Raspberry Pi 3159.ipt
- C:\Users\jferner\Downloads\raspberry-pi-3-model-b-reference-design-solidworks-cad-rpi-raspberrypi-raspberry-pi-1.snapshot.83\Solidworks Complete Assembly\Raspberry Pi 3160.ipt
- C:\Users\jferner\Downloads\raspberry-pi-3-model-b-reference-design-solidworks-cad-rpi-raspberrypi-raspberry-pi-1.snapshot.83\Solidworks Complete Assembly\Raspberry Pi 3161.ipt
- C:\Users\jferner\Downloads\raspberry-pi-3-model-b-reference-design-solidworks-cad-rpi-raspberrypi-raspberry-pi-1.snapshot.83\Solidworks Complete Assembly\Raspberry Pi 3162.ipt
- C:\Users\jferner\Downloads\raspberry-pi-3-model-b-reference-design-solidworks-cad-rpi-raspberrypi-raspberry-pi-1.snapshot.83\Solidworks Complete Assembly\Raspberry Pi 3163.ipt
- C:\Users\jferner\Downloads\raspberry-pi-3-model-b-reference-design-solidworks-cad-rpi-raspberrypi-raspberry-pi-1.snapshot.83\Solidworks Complete Assembly\Raspberry Pi 3164.ipt
- C:\Users\jferner\Downloads\raspberry-pi-3-model-b-reference-design-solidworks-cad-rpi-raspberrypi-raspberry-pi-1.snapshot.83\Solidworks Complete Assembly\Raspberry Pi 3165.ipt
- C:\Users\jferner\Downloads\raspberry-pi-3-model-b-reference-design-solidworks-cad-rpi-raspberrypi-raspberry-pi-1.snapshot.83\Solidworks Complete Assembly\Raspberry Pi 3166.ipt
- C:\Users\jferner\Downloads\raspberry-pi-3-model-b-reference-design-solidworks-cad-rpi-raspberrypi-raspberry-pi-1.snapshot.83\Solidworks Complete Assembly\Raspberry Pi 3167.ipt
- C:\Users\jferner\Downloads\raspberry-pi-3-model-b-reference-design-solidworks-cad-rpi-raspberrypi-raspberry-pi-1.snapshot.83\Solidworks Complete Assembly\Raspberry Pi 3168.ipt
- C:\Users\jferner\Downloads\raspberry-pi-3-model-b-reference-design-solidworks-cad-rpi-raspberrypi-raspberry-pi-1.snapshot.83\Solidworks Complete Assembly\Raspberry Pi 3169.ipt
- C:\Users\jferner\Downloads\raspberry-pi-3-model-b-reference-design-solidworks-cad-rpi-raspberrypi-raspberry-pi-1.snapshot.83\Solidworks Complete Assembly\Raspberry Pi 3170.ipt
- C:\Users\jferner\Downloads\raspberry-pi-3-model-b-reference-design-solidworks-cad-rpi-raspberrypi-raspberry-pi-1.snapshot.83\Solidworks Complete Assembly\Raspberry Pi 3171.ipt
- C:\Users\jferner\Downloads\raspberry-pi-3-model-b-reference-design-solidworks-cad-rpi-raspberrypi-raspberry-pi-1.snapshot.83\Solidworks Complete Assembly\Raspberry Pi 3276.ipt
- C:\Users\jferner\Downloads\raspberry-pi-3-model-b-reference-design-solidworks-cad-rpi-raspberrypi-raspberry-pi-1.snapshot.83\Solidworks Complete Assembly\Raspberry Pi 3277.ipt
- C:\Users\jferner\Downloads\raspberry-pi-3-model-b-reference-design-solidworks-cad-rpi-raspberrypi-raspberry-pi-1.snapshot.83\Solidworks Complete Assembly\Raspberry Pi 3278.ipt
- C:\Users\jferner\Downloads\raspberry-pi-3-model-b-reference-design-solidworks-cad-rpi-raspberrypi-raspberry-pi-1.snapshot.83\Solidworks Complete Assembly\Raspberry Pi 3279.ipt
- C:\Users\jferner\Downloads\raspberry-pi-3-model-b-reference-design-solidworks-cad-rpi-raspberrypi-raspberry-pi-1.snapshot.83\Solidworks Complete Assembly\Raspberry Pi 3280.ipt
- C:\Users\jferner\Downloads\raspberry-pi-3-model-b-reference-design-solidworks-cad-rpi-raspberrypi-raspberry-pi-1.snapshot.83\Solidworks Complete Assembly\Raspberry Pi 3281.ipt
- C:\Users\jferner\Downloads\raspberry-pi-3-model-b-reference-design-solidworks-cad-rpi-raspberrypi-raspberry-pi-1.snapshot.83\Solidworks Complete Assembly\Raspberry Pi 3282.ipt
- C:\Users\jferner\Downloads\raspberry-pi-3-model-b-reference-design-solidworks-cad-rpi-raspberrypi-raspberry-pi-1.snapshot.83\Solidworks Complete Assembly\Raspberry Pi 3283.ipt
- C:\Users\jferner\Downloads\raspberry-pi-3-model-b-reference-design-solidworks-cad-rpi-raspberrypi-raspberry-pi-1.snapshot.83\Solidworks Complete Assembly\Raspberry Pi 3284.ipt
- C:\Users\jferner\Downloads\raspberry-pi-3-model-b-reference-design-solidworks-cad-rpi-raspberrypi-raspberry-pi-1.snapshot.83\Solidworks Complete Assembly\Raspberry Pi 3285.ipt
- C:\Users\jferner\Downloads\raspberry-pi-3-model-b-reference-design-solidworks-cad-rpi-raspberrypi-raspberry-pi-1.snapshot.83\Solidworks Complete Assembly\Raspberry Pi 3286.ipt
- C:\Users\jferner\Downloads\raspberry-pi-3-model-b-reference-design-solidworks-cad-rpi-raspberrypi-raspberry-pi-1.snapshot.83\Solidworks Complete Assembly\Raspberry Pi 3287.ipt
- C:\Users\jferner\Downloads\raspberry-pi-3-model-b-reference-design-solidworks-cad-rpi-raspberrypi-raspberry-pi-1.snapshot.83\Solidworks Complete Assembly\Raspberry Pi 3288.ipt
- C:\Users\jferner\Downloads\raspberry-pi-3-model-b-reference-design-solidworks-cad-rpi-raspberrypi-raspberry-pi-1.snapshot.83\Solidworks Complete Assembly\Raspberry Pi 3289.ipt
- C:\Users\jferner\Downloads\raspberry-pi-3-model-b-reference-design-solidworks-cad-rpi-raspberrypi-raspberry-pi-1.snapshot.83\Solidworks Complete Assembly\Raspberry Pi 3290.ipt
- C:\Users\jferner\Downloads\raspberry-pi-3-model-b-reference-design-solidworks-cad-rpi-raspberrypi-raspberry-pi-1.snapshot.83\Solidworks Complete Assembly\Raspberry Pi 3291.ipt
- C:\Users\jferner\Downloads\raspberry-pi-3-model-b-reference-design-solidworks-cad-rpi-raspberrypi-raspberry-pi-1.snapshot.83\Solidworks Complete Assembly\Raspberry Pi 3292.ipt
- C:\Users\jferner\Downloads\raspberry-pi-3-model-b-reference-design-solidworks-cad-rpi-raspberrypi-raspberry-pi-1.snapshot.83\Solidworks Complete Assembly\Raspberry Pi 3293.ipt
- C:\Users\jferner\Downloads\raspberry-pi-3-model-b-reference-design-solidworks-cad-rpi-raspberrypi-raspberry-pi-1.snapshot.83\Solidworks Complete Assembly\Raspberry Pi 3294.ipt
- C:\Users\jferner\Downloads\raspberry-pi-3-model-b-reference-design-solidworks-cad-rpi-raspberrypi-raspberry-pi-1.snapshot.83\Solidworks Complete Assembly\Raspberry Pi 3295.ipt
- C:\Users\jferner\Downloads\raspberry-pi-3-model-b-reference-design-solidworks-cad-rpi-raspberrypi-raspberry-pi-1.snapshot.83\Solidworks Complete Assembly\Raspberry Pi 3296.ipt
- C:\Users\jferner\Downloads\raspberry-pi-3-model-b-reference-design-solidworks-cad-rpi-raspberrypi-raspberry-pi-1.snapshot.83\Solidworks Complete Assembly\Raspberry Pi 3297.ipt
- C:\Users\jferner\Downloads\raspberry-pi-3-model-b-reference-design-solidworks-cad-rpi-raspberrypi-raspberry-pi-1.snapshot.83\Solidworks Complete Assembly\Raspberry Pi 3298.ipt
- C:\Users\jferner\Downloads\raspberry-pi-3-model-b-reference-design-solidworks-cad-rpi-raspberrypi-raspberry-pi-1.snapshot.83\Solidworks Complete Assembly\Raspberry Pi 3299.ipt
- C:\Users\jferner\Downloads\raspberry-pi-3-model-b-reference-design-solidworks-cad-rpi-raspberrypi-raspberry-pi-1.snapshot.83\Solidworks Complete Assembly\Raspberry Pi 3300.ipt
- C:\Users\jferner\Downloads\raspberry-pi-3-model-b-reference-design-solidworks-cad-rpi-raspberrypi-raspberry-pi-1.snapshot.83\Solidworks Complete Assembly\Raspberry Pi 3301.ipt
- C:\Users\jferner\Downloads\raspberry-pi-3-model-b-reference-design-solidworks-cad-rpi-raspberrypi-raspberry-pi-1.snapshot.83\Solidworks Complete Assembly\Raspberry Pi 3302.ipt
- C:\Users\jferner\Downloads\raspberry-pi-3-model-b-reference-design-solidworks-cad-rpi-raspberrypi-raspberry-pi-1.snapshot.83\Solidworks Complete Assembly\Raspberry Pi 3303.ipt
- C:\Users\jferner\Downloads\raspberry-pi-3-model-b-reference-design-solidworks-cad-rpi-raspberrypi-raspberry-pi-1.snapshot.83\Solidworks Complete Assembly\Raspberry Pi 3304.ipt
- C:\Users\jferner\Downloads\raspberry-pi-3-model-b-reference-design-solidworks-cad-rpi-raspberrypi-raspberry-pi-1.snapshot.83\Solidworks Complete Assembly\Raspberry Pi 3305.ipt
- C:\Users\jferner\Downloads\raspberry-pi-3-model-b-reference-design-solidworks-cad-rpi-raspberrypi-raspberry-pi-1.snapshot.83\Solidworks Complete Assembly\Raspberry Pi 3306.ipt
- C:\Users\jferner\Downloads\raspberry-pi-3-model-b-reference-design-solidworks-cad-rpi-raspberrypi-raspberry-pi-1.snapshot.83\Solidworks Complete Assembly\Raspberry Pi 3307.ipt
- C:\Users\jferner\Downloads\raspberry-pi-3-model-b-reference-design-solidworks-cad-rpi-raspberrypi-raspberry-pi-1.snapshot.83\Solidworks Complete Assembly\Raspberry Pi 3308.ipt
- C:\Users\jferner\Downloads\raspberry-pi-3-model-b-reference-design-solidworks-cad-rpi-raspberrypi-raspberry-pi-1.snapshot.83\Solidworks Complete Assembly\Raspberry Pi 3309.ipt
- C:\Users\jferner\Downloads\raspberry-pi-3-model-b-reference-design-solidworks-cad-rpi-raspberrypi-raspberry-pi-1.snapshot.83\Solidworks Complete Assembly\Raspberry Pi 3310.ipt
- C:\Users\jferner\Downloads\raspberry-pi-3-model-b-reference-design-solidworks-cad-rpi-raspberrypi-raspberry-pi-1.snapshot.83\Solidworks Complete Assembly\Raspberry Pi 3311.ipt
- C:\Users\jferner\Downloads\raspberry-pi-3-model-b-reference-design-solidworks-cad-rpi-raspberrypi-raspberry-pi-1.snapshot.83\Solidworks Complete Assembly\Raspberry Pi 3312.ipt
- C:\Users\jferner\Downloads\raspberry-pi-3-model-b-reference-design-solidworks-cad-rpi-raspberrypi-raspberry-pi-1.snapshot.83\Solidworks Complete Assembly\Raspberry Pi 3313.ipt
- C:\Users\jferner\Downloads\raspberry-pi-3-model-b-reference-design-solidworks-cad-rpi-raspberrypi-raspberry-pi-1.snapshot.83\Solidworks Complete Assembly\Raspberry Pi 3314.ipt
- C:\Users\jferner\Downloads\raspberry-pi-3-model-b-reference-design-solidworks-cad-rpi-raspberrypi-raspberry-pi-1.snapshot.83\Solidworks Complete Assembly\Raspberry Pi 3315.ipt
- C:\Users\jferner\Downloads\raspberry-pi-3-model-b-reference-design-solidworks-cad-rpi-raspberrypi-raspberry-pi-1.snapshot.83\Solidworks Complete Assembly\Raspberry Pi 3316.ipt
- C:\Users\jferner\Downloads\raspberry-pi-3-model-b-reference-design-solidworks-cad-rpi-raspberrypi-raspberry-pi-1.snapshot.83\Solidworks Complete Assembly\Raspberry Pi 3317.ipt
- C:\Users\jferner\Downloads\raspberry-pi-3-model-b-reference-design-solidworks-cad-rpi-raspberrypi-raspberry-pi-1.snapshot.83\Solidworks Complete Assembly\Raspberry Pi 3318.ipt
- C:\Users\jferner\Downloads\raspberry-pi-3-model-b-reference-design-solidworks-cad-rpi-raspberrypi-raspberry-pi-1.snapshot.83\Solidworks Complete Assembly\Raspberry Pi 3319.ipt